# Autodesk Inventor assembly: 付け根_1
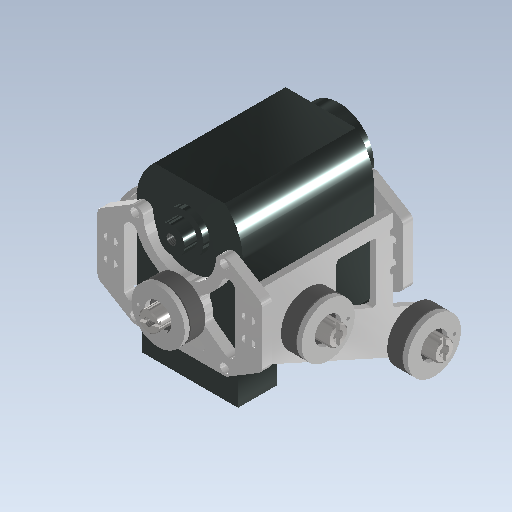
[picture p0: Inventor's stored thumbnail of the model, 512x512]
Saved by Autodesk Inventor 2020.4 (Build 244396000, 396)
## iProperties
Created: 2021-09-06
Part Number: 付け根_1
Document SubType Name: Assembly
Designer: Masato
Mass: 155.537 g
Surface Area: 333.044 cm^2
Volume: 75.5065 cm^3
Density: 2.05992 g/cm^3
Author: Masato
## Documents named in this file (11)
- C:\Users\Masato\Documents\Inventor\CIT Brains_Inventor\OpenPlatform_ver3_0\下半身\付け根\付け根_1.iam
- C:\Users\Masato\Documents\Inventor\CIT Brains_Inventor\OpenPlatform_ver3_0\下半身\付け根\付け根_メインフレーム_1.ipt
- C:\Users\Masato\Documents\Inventor\CIT Brains_Inventor\OpenPlatform_ver3_0\下半身\付け根\付け根_メインフレーム_6_1.ipt
- C:\Users\Masato\Documents\Inventor\CIT Brains_Inventor\OpenPlatform_ver3_0\Ready_Made\B3M11xx.ipt
- C:\Users\Masato\Documents\Inventor\CIT Brains_Inventor\OpenPlatform_ver3_0\Ready_Made\SLSBF6-39_5-M3-N3.ipt
- C:\Users\Masato\Documents\Inventor\CIT Brains_Inventor\OpenPlatform_ver3_0\Ready_Made\ARU-309_5S.ipt
- C:\Users\Masato\Documents\Inventor\CIT Brains_Inventor\OpenPlatform_ver3_0\Ready_Made\UUW-0312-10BH.ipt
- C:\Users\Masato\Documents\Inventor\CIT Brains_Inventor\OpenPlatform_ver3_0\Ready_Made\BRU-309_5S.ipt
- C:\Users\Masato\Documents\Inventor\CIT Brains_Inventor\OpenPlatform_ver3_0\Ready_Made\GSB-081605.ipt
- C:\Users\Masato\Documents\Inventor\CIT Brains_Inventor\OpenPlatform_ver3_0\Ready_Made\LFW-0815.ipt
- C:\Users\Masato\Documents\Inventor\CIT Brains_Inventor\OpenPlatform_ver3_0\Ready_Made\S3-07-3W.ipt
## Components (30 placed, 10 different names)
1. 付け根_メインフレーム_1:1 — メイト:1, メイト:2, フラッシュ:1, 挿入:11, 挿入:27, 挿入:28, 挿入:45
2. 付け根_メインフレーム_1:2 — メイト:3, メイト:4, フラッシュ:2, 挿入:12, 挿入:25, 挿入:26, 挿入:46
3. 付け根_メインフレーム_6_1:1 — 挿入:3, 挿入:4, 挿入:5, 挿入:6, メイト:1, メイト:2, フラッシュ:1, メイト:3, メイト:4, フラッシュ:2, 挿入:47, 挿入:49
4. 付け根_メインフレーム_6_1:2 — 挿入:7, 挿入:8, 挿入:9, 挿入:10, 挿入:50, 挿入:52
5. B3M11xx:1 — 挿入:3, 挿入:4, 挿入:5, 挿入:6, 挿入:7, 挿入:8, 挿入:9, 挿入:10, フラッシュ:6, メイト:8
6. SLSBF6-39_5-M3-N3:1 — 挿入:11, 挿入:12
7. ARU-309_5S:1 — 挿入:52
8. ARU-309_5S:2 — 挿入:49
9. UUW-0312-10BH:1 — 挿入:27, 挿入:35, 挿入:37
10. UUW-0312-10BH:2 — 挿入:28, 挿入:33, 挿入:38
11. UUW-0312-10BH:3 — 挿入:25, 挿入:36, 挿入:39
12. UUW-0312-10BH:4 — 挿入:26, 挿入:34, 挿入:40
13. BRU-309_5S:1 — 挿入:33
14. BRU-309_5S:2 — 挿入:34
15. BRU-309_5S:3 — 挿入:35
16. BRU-309_5S:4 — 挿入:36
17. GSB-081605:1 — 挿入:37, 挿入:41
18. GSB-081605:2 — 挿入:39, 挿入:44
19. GSB-081605:3 — 挿入:40, 挿入:43
20. GSB-081605:4 — 挿入:38, 挿入:42
21. LFW-0815:1 — 挿入:43
22. LFW-0815:2 — 挿入:44
23. LFW-0815:3 — 挿入:42
24. LFW-0815:4 — 挿入:41
25. S3-07-3W:1 — 挿入:45
26. S3-07-3W:2 — 挿入:46
27. GSB-081605:5 — 挿入:47, 挿入:48
28. LFW-0815:5 — 挿入:48
29. GSB-081605:6 — 挿入:50, 挿入:51
30. LFW-0815:6 — 挿入:51
## Relationships (42: Insert 34, Mate 5, Flush 3)
- 挿入:3 [Insert]: 付け根_メインフレーム_6_1:1 ↔ B3M11xx:1
- 挿入:4 [Insert]: 付け根_メインフレーム_6_1:1 ↔ B3M11xx:1
- 挿入:5 [Insert]: 付け根_メインフレーム_6_1:1 ↔ B3M11xx:1
- 挿入:6 [Insert]: 付け根_メインフレーム_6_1:1 ↔ B3M11xx:1
- 挿入:7 [Insert]: 付け根_メインフレーム_6_1:2 ↔ B3M11xx:1
- 挿入:8 [Insert]: 付け根_メインフレーム_6_1:2 ↔ B3M11xx:1
- 挿入:9 [Insert]: 付け根_メインフレーム_6_1:2 ↔ B3M11xx:1
- 挿入:10 [Insert]: 付け根_メインフレーム_6_1:2 ↔ B3M11xx:1
- メイト:1 [Mate] (0.01 mm): 付け根_メインフレーム_1:1 ↔ 付け根_メインフレーム_6_1:1
- メイト:2 [Mate] (0.01 mm): 付け根_メインフレーム_1:1 ↔ 付け根_メインフレーム_6_1:1
- フラッシュ:1 [Flush]: 付け根_メインフレーム_1:1 ↔ 付け根_メインフレーム_6_1:1
- メイト:3 [Mate] (0.01 mm): 付け根_メインフレーム_1:2 ↔ 付け根_メインフレーム_6_1:1
- メイト:4 [Mate] (0.01 mm): 付け根_メインフレーム_1:2 ↔ 付け根_メインフレーム_6_1:1
- フラッシュ:2 [Flush]: 付け根_メインフレーム_1:2 ↔ 付け根_メインフレーム_6_1:1
- 挿入:11 [Insert]: 付け根_メインフレーム_1:1 ↔ SLSBF6-39_5-M3-N3:1
- 挿入:12 [Insert]: 付け根_メインフレーム_1:2 ↔ SLSBF6-39_5-M3-N3:1
- 挿入:25 [Insert]: 付け根_メインフレーム_1:2 ↔ UUW-0312-10BH:3
- 挿入:26 [Insert]: 付け根_メインフレーム_1:2 ↔ UUW-0312-10BH:4
- 挿入:27 [Insert]: 付け根_メインフレーム_1:1 ↔ UUW-0312-10BH:1
- 挿入:28 [Insert]: 付け根_メインフレーム_1:1 ↔ UUW-0312-10BH:2
- 挿入:33 [Insert]: UUW-0312-10BH:2 ↔ BRU-309_5S:1
- 挿入:34 [Insert]: UUW-0312-10BH:4 ↔ BRU-309_5S:2
- フラッシュ:6 [Flush]: B3M11xx:1
- メイト:8 [Mate]: B3M11xx:1
- 挿入:35 [Insert]: UUW-0312-10BH:1 ↔ BRU-309_5S:3
- 挿入:36 [Insert]: UUW-0312-10BH:3 ↔ BRU-309_5S:4
- 挿入:37 [Insert]: UUW-0312-10BH:1 ↔ GSB-081605:1
- 挿入:38 [Insert]: UUW-0312-10BH:2 ↔ GSB-081605:4
- 挿入:39 [Insert]: UUW-0312-10BH:3 ↔ GSB-081605:2
- 挿入:40 [Insert]: UUW-0312-10BH:4 ↔ GSB-081605:3
- 挿入:41 [Insert]: GSB-081605:1 ↔ LFW-0815:4
- 挿入:42 [Insert]: GSB-081605:4 ↔ LFW-0815:3
- 挿入:43 [Insert]: GSB-081605:3 ↔ LFW-0815:1
- 挿入:44 [Insert]: GSB-081605:2 ↔ LFW-0815:2
- 挿入:45 [Insert]: 付け根_メインフレーム_1:1 ↔ S3-07-3W:1
- 挿入:46 [Insert]: 付け根_メインフレーム_1:2 ↔ S3-07-3W:2
- 挿入:47 [Insert]: 付け根_メインフレーム_6_1:1 ↔ GSB-081605:5
- 挿入:48 [Insert]: GSB-081605:5 ↔ LFW-0815:5
- 挿入:49 [Insert]: 付け根_メインフレーム_6_1:1 ↔ ARU-309_5S:2
- 挿入:50 [Insert]: 付け根_メインフレーム_6_1:2 ↔ GSB-081605:6
- 挿入:51 [Insert]: GSB-081605:6 ↔ LFW-0815:6
- 挿入:52 [Insert]: 付け根_メインフレーム_6_1:2 ↔ ARU-309_5S:1
